# Autodesk Inventor assembly: RevSingleStage
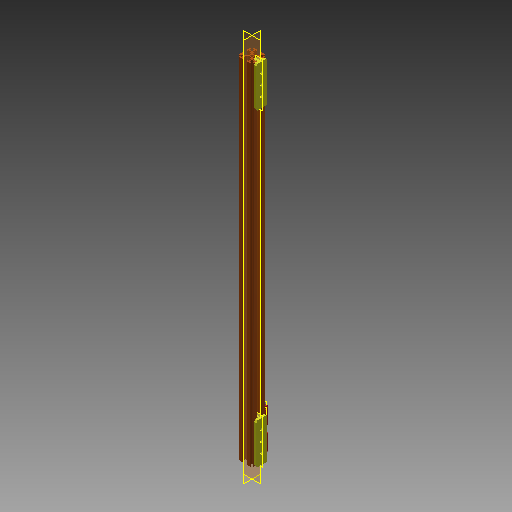
[picture p0: Inventor's stored thumbnail of the model, 512x512]
Saved by Autodesk Inventor 2018 (Build 220112000, 112)
## iProperties
Created: 2017-11-25
Part Number: RevSingleStage
Document SubType Name: Assembly
Designer: ball
Author: ball
## Documents named in this file (4)
- C:\FTC\FTC8863CAD\2017Robot\RevSingleStage.iam
- C:\FTC\FTC8863CAD\RevRobotics\REV-41-1017_15mm_extrusion_17.875in.ipt
- C:\FTC\FTC8863CAD\RevRobotics\REV-41-1095.ipt
- C:\FTC\FTC8863CAD\RevRobotics\REV-41-1094.ipt
## Components (4 placed, 3 different names)
1. REV-41-1017_15mm_extrusion_17.875in:2 — Mate:1, Mate:2, Flush:3, Mate:3, Mate:4, Flush:4, Mate:5, Mate:6, Flush:5
2. REV-41-1095:1 — Mate:1, Mate:2, Flush:3
3. REV-41-1095:2 — Mate:3, Mate:4, Flush:4
4. REV-41-1094:1 — Mate:5, Mate:6, Flush:5
## Relationships (9: Mate 6, Flush 3)
- Mate:1: REV-41-1017_15mm_extrusion_17.875in:2 ↔ REV-41-1095:1
- Mate:2: REV-41-1017_15mm_extrusion_17.875in:2 ↔ REV-41-1095:1
- Flush:3: REV-41-1017_15mm_extrusion_17.875in:2 ↔ REV-41-1095:1
- Mate:3: REV-41-1017_15mm_extrusion_17.875in:2 ↔ REV-41-1095:2
- Mate:4: REV-41-1017_15mm_extrusion_17.875in:2 ↔ REV-41-1095:2
- Flush:4: REV-41-1017_15mm_extrusion_17.875in:2 ↔ REV-41-1095:2
- Mate:5: REV-41-1017_15mm_extrusion_17.875in:2 ↔ REV-41-1094:1
- Mate:6: REV-41-1017_15mm_extrusion_17.875in:2 ↔ REV-41-1094:1
- Flush:5: REV-41-1017_15mm_extrusion_17.875in:2 ↔ REV-41-1094:1
